# Autodesk Inventor assembly: TorsoActuator
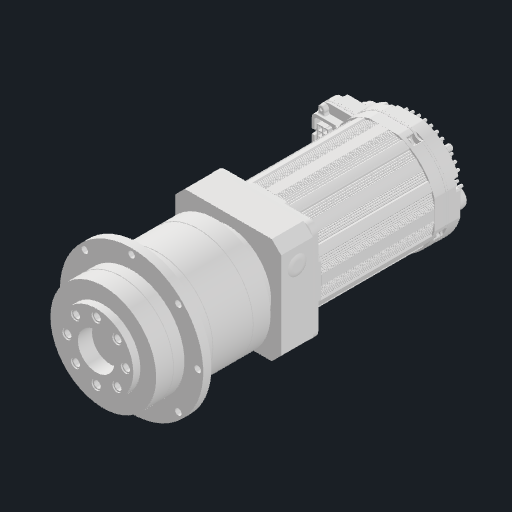
[picture p0: Inventor's stored thumbnail of the model, 512x512]
Saved by Autodesk Inventor 2025.2 (Build 292293000, 293)
## iProperties
Created: 2025-02-09
Part Number: TorsoActuator
Document SubType Name: Assembly
Designer: LattePanda
Author: LattePanda
## Documents named in this file (3)
- C:\Users\valer\Desktop\str1ker\cad\external\TorsoActuator\TorsoActuator.iam
- C:\Users\valer\Desktop\str1ker\cad\external\TorsoActuator\TorsoGearbox.ipt
- C:\Users\valer\Desktop\str1ker\cad\external\TorsoActuator\TorsoMotor.ipt
## Components (2 placed, 2 different names)
1. TorsoGearbox:1 — Flush:1, Mate:1, Angle:1, Mate:2, Mate:3, Mate:4
2. TorsoMotor:1 — Mate:2, Mate:3, Mate:4
## Relationships (6: Mate 4, Flush 1, Angle 1)
- Flush:1: TorsoGearbox:1
- Mate:1: TorsoGearbox:1
- Angle:1 (0 deg): TorsoGearbox:1
- Mate:2: TorsoGearbox:1 ↔ TorsoMotor:1
- Mate:3: TorsoGearbox:1 ↔ TorsoMotor:1
- Mate:4: TorsoGearbox:1 ↔ TorsoMotor:1
